# Autodesk Inventor assembly: plantiBox
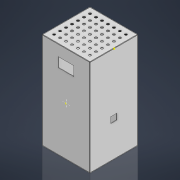
[picture p0: Inventor's stored thumbnail of the model, 180x180]
Saved by Autodesk Inventor 2021 (Build 250183000, 183)
## iProperties
Created: 2021-03-25
Part Number: plantiBox
Document SubType Name: Assembly
Designer: noori
Author: noori
## Documents named in this file (6)
- C:\Users\Public\Documents\Autodesk\Inventor 2021\planti\plantiBox.iam
- C:\Users\Public\Documents\Autodesk\Inventor 2021\planti\bottom.ipt
- C:\Users\Public\Documents\Autodesk\Inventor 2021\planti\left.ipt
- C:\Users\Public\Documents\Autodesk\Inventor 2021\planti\back.ipt
- C:\Users\Public\Documents\Autodesk\Inventor 2021\planti\front.ipt
- C:\Users\Public\Documents\Autodesk\Inventor 2021\planti\top.ipt
## Components (6 placed, 5 different names)
1. bottom:1 — Mate:1, Flush:1, Flush:2, Mate:2, Flush:3, Flush:4, Mate:3, Flush:5, Mate:4, Flush:8
2. left:2 — Mate:3, Flush:5, Flush:6, Mate:5
3. back:1 — Mate:1, Flush:1, Flush:2, Flush:6
4. front:1 — Mate:2, Flush:3, Flush:4, Flush:7, Flush:10
5. left:3 — Mate:4, Flush:7, Flush:8, Flush:9, Flush:11
6. top:1 — Mate:5, Flush:9, Flush:10, Flush:11
## Relationships (16: Flush 11, Mate 5)
- Mate:1: bottom:1 ↔ back:1
- Flush:1: bottom:1 ↔ back:1
- Flush:2: bottom:1 ↔ back:1
- Mate:2: bottom:1 ↔ front:1
- Flush:3: bottom:1 ↔ front:1
- Flush:4: bottom:1 ↔ front:1
- Mate:3: bottom:1 ↔ left:2
- Flush:5: bottom:1 ↔ left:2
- Flush:6: left:2 ↔ back:1
- Mate:4: bottom:1 ↔ left:3
- Flush:7: front:1 ↔ left:3
- Flush:8: bottom:1 ↔ left:3
- Mate:5: left:2 ↔ top:1
- Flush:9: left:3 ↔ top:1
- Flush:10: front:1 ↔ top:1
- Flush:11: left:3 ↔ top:1
